# Autodesk Inventor assembly: VersaPlanetary 500 Hex 1 stage
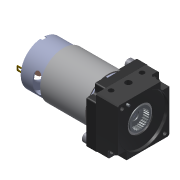
[picture p0: Inventor's stored thumbnail of the model, 180x180]
Saved by Autodesk Inventor 2013 (Build 170138000, 138)
## iProperties
Created: 2013-12-15
Part Number: VersaPlanetary 500 Hex 1 stage
Document SubType Name: Assembly
Designer: Nemo
Author: Nemo
## Documents named in this file (11)
- \\lmss\students\Robotics\CAD Files\COTS Parts\VersaPlanetary\VersaPlanetary AM-9015 Input.iam
- \\lmss\students\Robotics\CAD Files\COTS Parts\VersaPlanetary\Components\VersaPlanetary Case Motor Side.ipt
- \\lmss\students\Robotics\CAD Files\COTS Parts\VersaPlanetary\Components\VersaPlanetary Shaft Holder.ipt
- \\lmss\students\Robotics\CAD Files\COTS Parts\Bearings - VexPro\Radial Bearing - 17mm x 26mm x 5mm.ipt
- \\lmss\students\Robotics\CAD Files\COTS Parts\VersaPlanetary\Components\VersaPlanetary RS550 shaft piece.ipt
- \\lmss\students\Robotics\CAD Files\COTS Parts\Fasteners\8-32 SHCS x500.ipt
- \\lmss\students\Robotics\CAD Files\COTS Parts\VersaPlanetary\Components\VersaPlanetary shaft holder clip ring.ipt
- \\lmss\students\Robotics\CAD Files\COTS Parts\VersaPlanetary\Components\VersaPlanetary pin.ipt
- \\lmss\students\Robotics\CAD Files\COTS Parts\Fasteners\M4 SHCS x10.ipt
- \\lmss\students\Robotics\CAD Files\COTS Parts\Motors\AndyMark 9015 Motor AM-0912.ipt
- \\lmss\students\Robotics\CAD Files\COTS Parts\VersaPlanetary\Components\VersaPlanetary Mount Plate - AM-9015.ipt
## Components (12 placed, 10 different names)
1. VersaPlanetary Case Motor Side:1 — Mate:1, Mate:2, Insert:5, Mate:8, Mate:10, Mate:11, Flush:2, Mate:12, Mate:16, Flush:3, Flush:4
2. VersaPlanetary Shaft Holder:1 — Mate:3, Mate:4, Mate:5, Flush:1, Insert:4
3. Radial Bearing - 17mm x 26mm x 5mm:1 — Mate:1, Mate:2, Mate:3, Mate:4
4. VersaPlanetary RS550 shaft piece:1 — Mate:5, Flush:1
5. 8-32 SHCS x500:1 — Mate:8, Mate:13
6. 8-32 SHCS x500:2 — Mate:10, Mate:14
7. VersaPlanetary shaft holder clip ring:1 — Insert:4
8. VersaPlanetary pin:1 — Insert:5
9. M4 SHCS x10:1 — Insert:6
10. M4 SHCS x10:2 — Insert:7
11. AndyMark 9015 Motor AM-0912:1 — Insert:8, Mate:15
12. VersaPlanetary Mount Plate - AM-9015:1 — Mate:11, Flush:2, Mate:12, Mate:13, Mate:14, Insert:6, Insert:7, Insert:8, Mate:15
## Relationships (22: Mate 13, Insert 5, Flush 4)
- Mate:1: VersaPlanetary Case Motor Side:1 ↔ Radial Bearing - 17mm x 26mm x 5mm:1
- Mate:2: VersaPlanetary Case Motor Side:1 ↔ Radial Bearing - 17mm x 26mm x 5mm:1
- Mate:3: VersaPlanetary Shaft Holder:1 ↔ Radial Bearing - 17mm x 26mm x 5mm:1
- Mate:4: VersaPlanetary Shaft Holder:1 ↔ Radial Bearing - 17mm x 26mm x 5mm:1
- Mate:5: VersaPlanetary Shaft Holder:1 ↔ VersaPlanetary RS550 shaft piece:1
- Flush:1: VersaPlanetary Shaft Holder:1 ↔ VersaPlanetary RS550 shaft piece:1
- Insert:4: VersaPlanetary Shaft Holder:1 ↔ VersaPlanetary shaft holder clip ring:1
- Insert:5: VersaPlanetary Case Motor Side:1 ↔ VersaPlanetary pin:1
- Mate:8: VersaPlanetary Case Motor Side:1 ↔ 8-32 SHCS x500:1
- Mate:10: VersaPlanetary Case Motor Side:1 ↔ 8-32 SHCS x500:2
- Mate:11: VersaPlanetary Case Motor Side:1 ↔ VersaPlanetary Mount Plate - AM-9015:1
- Flush:2: VersaPlanetary Case Motor Side:1 ↔ VersaPlanetary Mount Plate - AM-9015:1
- Mate:12: VersaPlanetary Case Motor Side:1 ↔ VersaPlanetary Mount Plate - AM-9015:1
- Mate:13: 8-32 SHCS x500:1 ↔ VersaPlanetary Mount Plate - AM-9015:1
- Mate:14: 8-32 SHCS x500:2 ↔ VersaPlanetary Mount Plate - AM-9015:1
- Insert:6: M4 SHCS x10:1 ↔ VersaPlanetary Mount Plate - AM-9015:1
- Insert:7: M4 SHCS x10:2 ↔ VersaPlanetary Mount Plate - AM-9015:1
- Insert:8: AndyMark 9015 Motor AM-0912:1 ↔ VersaPlanetary Mount Plate - AM-9015:1
- Mate:15: AndyMark 9015 Motor AM-0912:1 ↔ VersaPlanetary Mount Plate - AM-9015:1
- Mate:16: VersaPlanetary Case Motor Side:1
- Flush:3: VersaPlanetary Case Motor Side:1
- Flush:4: VersaPlanetary Case Motor Side:1
